# Autodesk Inventor assembly: Laser Mount + Clamp
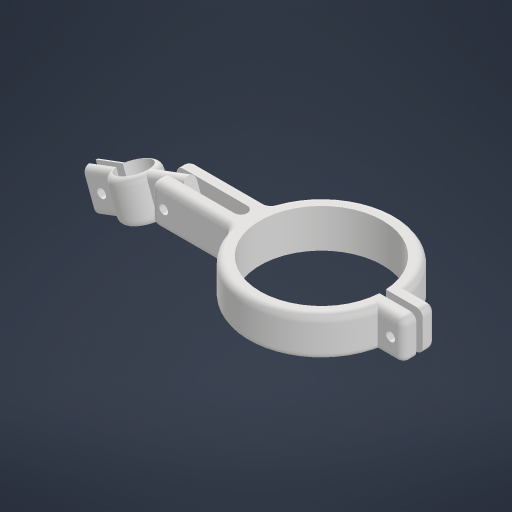
[picture p0: Inventor's stored thumbnail of the model, 512x512]
Saved by Autodesk Inventor 2024.1 (Build 281209000, 209)
## iProperties
Created: 2024-11-18
Part Number: Laser Mount + Clamp
Document SubType Name: Assembly
Designer: Designer
Author: Designer
## Documents named in this file (5)
- C:\Users\Designer\Desktop\optics\Traj\Laser Mount + Clamp.iam
- C:\Users\Designer\Desktop\optics\Traj\Clamp.ipt
- C:\Users\Designer\Desktop\optics\Traj\Laser Mount.ipt
- C:\Users\Designer\Documents\Inventor\Content Center Files\R2024\VEX-CAD-Inventor-main\Structure\Hardware\Screw Steel - Star\SScrew Star Smooth .250.ipt
- C:\Users\Designer\Documents\Inventor\Content Center Files\R2024\VEX-CAD-Inventor-main\Structure\Hardware\Screw Steel - Star.ipt
## Components (5 placed, 3 different names)
1. Clamp:1 — Rotational:1, Rigid:1, Rigid:2
2. Laser Mount:1 — Rotational:1, Rigid:3
3. SScrew Star Smooth .250:1 — Rigid:3
4. SScrew Star Smooth .250:2 — Rigid:2
5. SScrew Star Smooth .250:3 — Rigid:1
## Relationships (4: WeldJoint 3, RevoluteJoint 1)
- Rotational:1 [RevoluteJoint]: Clamp:1 ↔ Laser Mount:1
- Rigid:1 [WeldJoint]: Clamp:1 ↔ SScrew Star Smooth .250:3
- Rigid:2 [WeldJoint]: Clamp:1 ↔ SScrew Star Smooth .250:2
- Rigid:3 [WeldJoint]: Laser Mount:1 ↔ SScrew Star Smooth .250:1
